# Autodesk Inventor assembly: Konstruktion_schuh_print_004
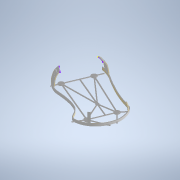
[picture p0: Inventor's stored thumbnail of the model, 180x180]
Saved by Autodesk Inventor 2020.2 (Build 242310000, 310)
## iProperties
Created: 2020-03-13
Part Number: Konstruktion_schuh_print_004
Document SubType Name: Assembly
Designer: Mara
Author: Mara
## Documents named in this file (3)
- C:\Users\Mara\Masterarbeit_CAD\Konstruktion_schuh_print_004.iam
- C:\Users\Mara\Masterarbeit_CAD\Grundform_Oben.ipt
- C:\Users\Mara\Masterarbeit_CAD\Grundform_Boden.ipt
## Components (2 placed, 2 different names)
1. Grundform_Oben:1 — Mate:1
2. Grundform_Boden:1 — Mate:1
## Relationships (1: Mate 1)
- Mate:1: Grundform_Oben:1 ↔ Grundform_Boden:1
